# Autodesk Inventor assembly: Mechanics Assembly
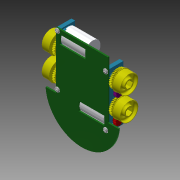
[picture p0: Inventor's stored thumbnail of the model, 180x180]
Saved by Autodesk Inventor 2014 (Build 180170000, 170)
## iProperties
Created: 2013-09-11
Part Number: Mechanics Assembly
Document SubType Name: Assembly
Designer: Brandon
Author: Brandon
## Documents named in this file (11)
- E:\ENGINEERING\IEEEUCR-MM-2014\HARDWARE\REFERENCE_MOUSE_V1\3D\Mechanics Assembly.iam
- E:\ENGINEERING\IEEEUCR-MM-2014\HARDWARE\REFERENCE_MOUSE_V1\3D\Wheel.ipt
- E:\ENGINEERING\IEEEUCR-MM-2014\HARDWARE\REFERENCE_MOUSE_V1\3D\Wheel2Wheel.ipt
- E:\ENGINEERING\IEEEUCR-MM-2014\HARDWARE\REFERENCE_MOUSE_V1\3D\Wheel_MIR.ipt
- E:\ENGINEERING\IEEEUCR-MM-2014\HARDWARE\REFERENCE_MOUSE_V1\3D\mount.ipt
- E:\ENGINEERING\IEEEUCR-MM-2014\HARDWARE\REFERENCE_MOUSE_V1\3D\gear motor.ipt
- E:\ENGINEERING\IEEEUCR-MM-2014\HARDWARE\REFERENCE_MOUSE_V1\3D\idler shaft.ipt
- E:\ENGINEERING\IEEEUCR-MM-2014\HARDWARE\REFERENCE_MOUSE_V1\3D\PCB.ipt
- E:\ENGINEERING\IEEEUCR-MM-2014\HARDWARE\REFERENCE_MOUSE_V1\3D\motor.ipt
- E:\ENGINEERING\IEEEUCR-MM-2014\HARDWARE\REFERENCE_MOUSE_V1\3D\IMPORTED COMPONENTS\7804K129\7804K129.IPT
- E:\engineering\IEEEUCR-MM-2014\hardware\Reference_Mouse_v1\3D\IMPORTED COMPONENTS\92005A076\92005A076.IPT
## Components (22 placed, 19 different names)
1. LF Wheel — Rotation:3, Rotational:2, Rotation:5
2. Left Idler — Mate:1, Rotation:3, Rotational:3, Rotation:4
3. LB Wheel — Rotational:1, Rotation:4
4. Left Mount — Rotational:1, Rotational:2, Rotational:3, Rotational:4, Flush:2, Mate:5, Mate:8, Mate:9, Angle:1, Insert:1, Mate:22, Mate:23, Mate:24, Insert:3, Insert:4
5. Left Motor Output — Rotational:4, Rotation:5
6. RB Wheel
7. Right Idler
8. RF Wheel
9. Right Mount — Mate:3, Mate:6, Mate:7, Mate:10, Mate:18, Insert:2, Mate:21, Mate:25, Mate:26, Insert:5, Insert:6
10. Right Motor Output
11. Idler Shaft — Mate:14, Mate:15, Mate:16, Mate:17
12. PCB — Flush:3, Mate:19, Mate:20, Mate:23, Mate:24, Mate:25, Mate:26, Insert:7, Insert:8, Insert:9, Insert:10
13. L motor — Insert:1, Mate:22
14. R motor — Insert:2, Mate:21
15. LF Bearing — Insert:3
16. RF Bearing — Insert:5
17. RB Bearing — Insert:6
18. LB Bearing — Insert:4
19. 92005A076:1 — Insert:7
20. 92005A076:2 — Insert:10
21. 92005A076:3 — Insert:9
22. 92005A076:4 — Insert:8
## Relationships (51: Mate 24, Insert 10, RevoluteJoint 8, RelateRotation 6, Flush 2, Angle 1)
- Mate:1: Left Idler
- Rotation:3 [RelateRotation] (0.667 ul): LF Wheel ↔ Left Idler
- Rotational:1 [RevoluteJoint]: LB Wheel ↔ Left Mount
- Rotational:2 [RevoluteJoint]: LF Wheel ↔ Left Mount
- Rotational:3 [RevoluteJoint] (-1.25 mm): Left Idler ↔ Left Mount
- Rotation:4 [RelateRotation] (0.6667 ul): Left Idler ↔ LB Wheel
- Rotational:4 [RevoluteJoint] (0.2 mm): Left Mount ↔ Left Motor Output
- Rotation:5 [RelateRotation] (2 ul): LF Wheel ↔ Left Motor Output
- Flush:2 (-24.5 mm): Left Mount
- [RelateRotation] (0.667 ul): RB Wheel ↔ Right Idler
- [RevoluteJoint]: RF Wheel ↔ Right Mount
- [RevoluteJoint]: RB Wheel ↔ Right Mount
- [RevoluteJoint] (-1.25 mm): Right Idler ↔ Right Mount
- [RelateRotation] (0.6667 ul): Right Idler ↔ RF Wheel
- [RevoluteJoint] (0.2 mm): Right Mount ↔ Right Motor Output
- [RelateRotation] (2 ul): RB Wheel ↔ Right Motor Output
- Mate:3 (24.5 mm): Right Mount
- Mate:5: Left Mount
- Mate:6: Right Mount
- Mate:7 (4 mm): Right Mount
- Mate:8 (4 mm): Left Mount
- Mate:9: Left Mount
- Mate:10: Right Mount
- Mate:11
- Mate:12
- Mate:13
- Mate:14: Idler Shaft
- Mate:15: Idler Shaft
- Mate:16: Idler Shaft
- Mate:17: Idler Shaft
- Mate:18: Right Mount
- Angle:1 (0 deg): Left Mount
- Flush:3: PCB
- Mate:19 (-14 mm): PCB
- Mate:20: PCB
- Insert:1: Left Mount ↔ L motor
- Insert:2: Right Mount ↔ R motor
- Mate:21: Right Mount ↔ R motor
- Mate:22: Left Mount ↔ L motor
- Mate:23: Left Mount ↔ PCB
- Mate:24: Left Mount ↔ PCB
- Mate:25: Right Mount ↔ PCB
- Mate:26: Right Mount ↔ PCB
- Insert:3 (0.1 mm): Left Mount ↔ LF Bearing
- Insert:4 (0.1 mm): Left Mount ↔ LB Bearing
- Insert:5 (0.1 mm): Right Mount ↔ RF Bearing
- Insert:6 (0.1 mm): Right Mount ↔ RB Bearing
- Insert:7: PCB ↔ 92005A076:1
- Insert:8: PCB ↔ 92005A076:4
- Insert:9: PCB ↔ 92005A076:3
- Insert:10: PCB ↔ 92005A076:2
## Named parameters: d62_d57 = 0.2 mm, d63_d58 = -4.554369 deg, d64_d59 = 2, d65_d35 = 0 mm, d66_d36 = 61.162763 deg, d67_d39 = 0 mm, d68_d40 = -28.868955 deg, d69_d47 = -1.25 mm, d70_d48 = 9.663939 deg, d71_d55 = 0.666667, d72_d9 = 0.667
